# Autodesk Inventor assembly: case1
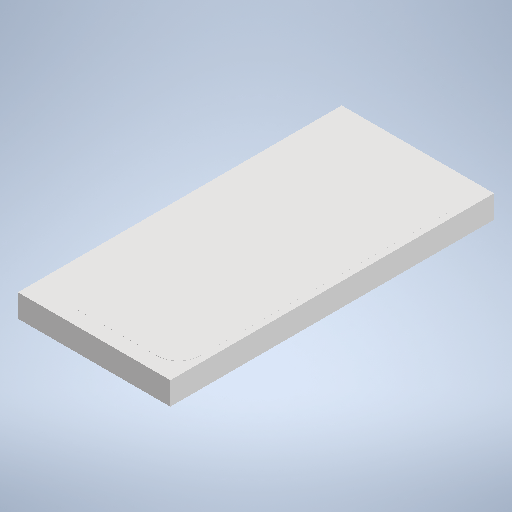
[picture p0: Inventor's stored thumbnail of the model, 512x512]
Saved by Autodesk Inventor 2025.2 (Build 292293000, 293)
## iProperties
Created: 2025-05-31
Part Number: case1
Document SubType Name: Assembly
Designer: mahhy
Author: mahhy
## Documents named in this file (3)
- D:\mahhy\個人用\設計データ\スマホケース\case1.iam
- D:\mahhy\個人用\設計データ\スマホケース\case.ipt
- D:\mahhy\個人用\設計データ\スマホケース\smartphone.ipt
## Components (2 placed, 2 different names)
1. case:1 — フラッシュ:1, リジッド:1
2. smartphone:1 — フラッシュ:1, リジッド:1
## Relationships (2: Flush 1, WeldJoint 1)
- フラッシュ:1 [Flush]: case:1 ↔ smartphone:1
- リジッド:1 [WeldJoint]: case:1 ↔ smartphone:1
